# Autodesk Inventor assembly: Hip
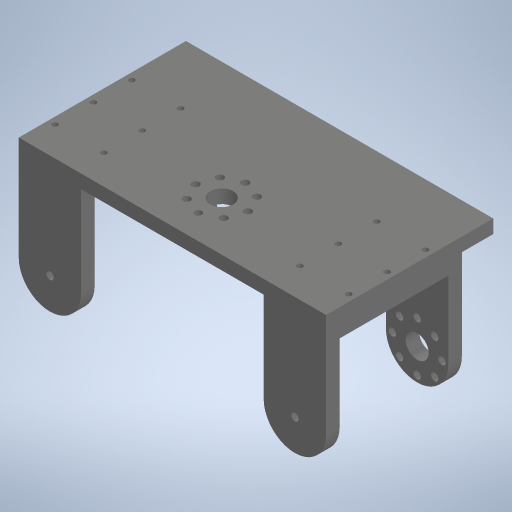
[picture p0: Inventor's stored thumbnail of the model, 512x512]
Saved by Autodesk Inventor 2024.3 (Build 283343000, 343)
## iProperties
Created: 2024-09-18
Part Number: Hip
Document SubType Name: Assembly
Designer: 구지현
Author: 구지현
## Documents named in this file (3)
- C:\Users\구지현\Desktop\19th_intern_kdy_robot\부품\Lower_Body\Hip\Hip.iam
- C:\Users\구지현\Desktop\19th_intern_kdy_robot\부품\Lower_Body\Hip\Hip_Body_Connection_Parts.ipt
- C:\Users\구지현\Desktop\19th_intern_kdy_robot\부품\Lower_Body\Hip\Hip_Leg_Connection_Parts.ipt
## Components (3 placed, 2 different names)
1. Hip_Body_Connection_Parts:1 — 삽입:1, 삽입:2, 삽입:3, 삽입:10, 삽입:11, 삽입:12, 삽입:13, 삽입:14, 삽입:15, 플러쉬:1, 플러쉬:2, 삽입:16, 삽입:17, 삽입:18, 삽입:19, 삽입:20, 삽입:21
2. Hip_Leg_Connection_Parts:1 — 삽입:1, 삽입:2, 삽입:3, 삽입:10, 삽입:11, 삽입:12, 삽입:13, 삽입:14, 삽입:15
3. Hip_Leg_Connection_Parts:2 — 삽입:16, 삽입:17, 삽입:18, 삽입:19, 삽입:20, 삽입:21
## Relationships (17: Insert 15, Flush 2)
- 삽입:1 [Insert]: Hip_Body_Connection_Parts:1 ↔ Hip_Leg_Connection_Parts:1
- 삽입:2 [Insert]: Hip_Body_Connection_Parts:1 ↔ Hip_Leg_Connection_Parts:1
- 삽입:3 [Insert]: Hip_Body_Connection_Parts:1 ↔ Hip_Leg_Connection_Parts:1
- 삽입:10 [Insert]: Hip_Body_Connection_Parts:1 ↔ Hip_Leg_Connection_Parts:1
- 삽입:11 [Insert]: Hip_Body_Connection_Parts:1 ↔ Hip_Leg_Connection_Parts:1
- 삽입:12 [Insert]: Hip_Body_Connection_Parts:1 ↔ Hip_Leg_Connection_Parts:1
- 삽입:13 [Insert]: Hip_Body_Connection_Parts:1 ↔ Hip_Leg_Connection_Parts:1
- 삽입:14 [Insert]: Hip_Body_Connection_Parts:1 ↔ Hip_Leg_Connection_Parts:1
- 삽입:15 [Insert]: Hip_Body_Connection_Parts:1 ↔ Hip_Leg_Connection_Parts:1
- 플러쉬:1 [Flush]: Hip_Body_Connection_Parts:1
- 플러쉬:2 [Flush]: Hip_Body_Connection_Parts:1
- 삽입:16 [Insert]: Hip_Body_Connection_Parts:1 ↔ Hip_Leg_Connection_Parts:2
- 삽입:17 [Insert]: Hip_Body_Connection_Parts:1 ↔ Hip_Leg_Connection_Parts:2
- 삽입:18 [Insert]: Hip_Body_Connection_Parts:1 ↔ Hip_Leg_Connection_Parts:2
- 삽입:19 [Insert]: Hip_Body_Connection_Parts:1 ↔ Hip_Leg_Connection_Parts:2
- 삽입:20 [Insert]: Hip_Body_Connection_Parts:1 ↔ Hip_Leg_Connection_Parts:2
- 삽입:21 [Insert]: Hip_Body_Connection_Parts:1 ↔ Hip_Leg_Connection_Parts:2
